# Autodesk Inventor assembly: MonoFilamentSpool22mm
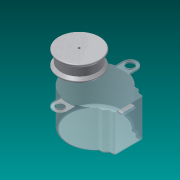
[picture p0: Inventor's stored thumbnail of the model, 180x180]
Saved by Autodesk Inventor 2013 (Build 170138000, 138)
## iProperties
Created: 2013-08-18
Part Number: MonoFilamentSpool22mm
Document SubType Name: Assembly
Designer: Sawaiz
Author: Sawaiz
## Documents named in this file (3)
- S:\Sawaiz\Documents\3D Modeling\Inventor\PolarGraph\MonoFilamentSpool22mm.iam
- S:\Sawaiz\Documents\3D Modeling\Inventor\PolarGraph\Stepper Motor 28BYJ-48.ipt
- S:\Sawaiz\Documents\3D Modeling\Inventor\PolarGraph\22mm Spool.ipt
## Components (2 placed, 2 different names)
1. Stepper Motor 28BYJ-48:1 — Mate:1, Mate:2
2. 22mm Spool:1 — Mate:1, Mate:2
## Relationships (2: Mate 2)
- Mate:1: Stepper Motor 28BYJ-48:1 ↔ 22mm Spool:1
- Mate:2: Stepper Motor 28BYJ-48:1 ↔ 22mm Spool:1
